# Autodesk Inventor assembly: PotHolderAssembly
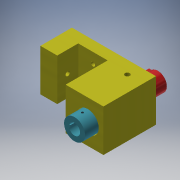
[picture p0: Inventor's stored thumbnail of the model, 180x180]
Saved by Autodesk Inventor 2018.2 (Build 222227000, 227)
## iProperties
Created: 2018-02-27
Part Number: PotHolderAssembly
Document SubType Name: Assembly
Designer: steele
Author: steele
## Documents named in this file (4)
- D:\snobotics\CAD-Development\robSteele\2018-FRC\Arm\PotHolderAssembly.iam
- D:\snobotics\CAD-Development\robSteele\2018-FRC\Arm\blockToSupportShaftAndPot.ipt
- D:\snobotics\CAD-Development\robSteele\2018-FRC\Arm\ShaftToConnectPotToMotor.ipt
- D:\snobotics\CAD-Development\robSteele\2018-FRC\Arm\10 turn potentiometer.ipt
## Components (3 placed, 3 different names)
1. blockToSupportShaftAndPot:1 — Insert:3
2. ShaftToConnectPotToMotor:1 — Insert:2, Insert:3
3. 10 turn potentiometer:1 — Insert:2
## Relationships (2: Insert 2)
- Insert:2 (1.27 mm): ShaftToConnectPotToMotor:1 ↔ 10 turn potentiometer:1
- Insert:3: blockToSupportShaftAndPot:1 ↔ ShaftToConnectPotToMotor:1
